# Autodesk Inventor assembly: 8 ball cable roller assembly
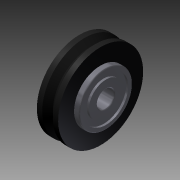
[picture p0: Inventor's stored thumbnail of the model, 180x180]
Saved by Autodesk Inventor 2012 (Build 160160000, 160)
## iProperties
Created: 2013-12-03
Part Number: 8 ball cable roller assembly
Document SubType Name: Assembly
Designer: Bryce
Author: Bryce
## Documents named in this file (3)
- C:\Users\Bryce\Dropbox\Inventor Design Project Files\Independent Swerves\Inventor 2012\8 ball cable roller assembly.iam
- C:\Users\Bryce\Dropbox\Inventor Design Project Files\Independent Swerves\Inventor 2012\8 ball cable roller bearing.ipt
- C:\Users\Bryce\Dropbox\Inventor Design Project Files\Independent Swerves\Inventor 2012\8 ball cable roller.ipt
## Components (2 placed, 2 different names)
1. 8 ball cable roller bearing:1 — Mate:1, Flush:1
2. 8 ball cable roller:1 — Mate:1, Flush:1
## Relationships (2: Mate 1, Flush 1)
- Mate:1: 8 ball cable roller bearing:1 ↔ 8 ball cable roller:1
- Flush:1 (-1.5875 mm): 8 ball cable roller bearing:1 ↔ 8 ball cable roller:1
